# Autodesk Inventor assembly: SUBWashChamber
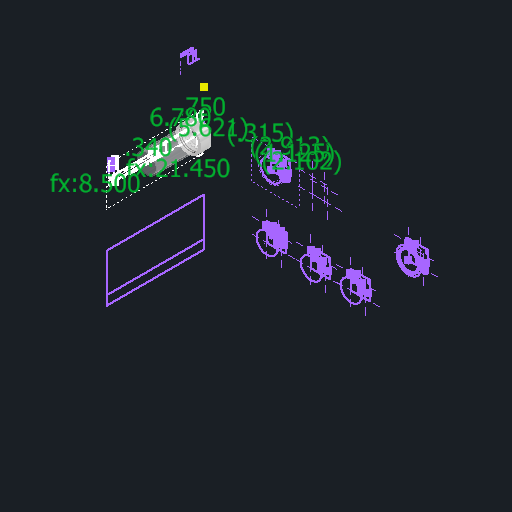
[picture p0: Inventor's stored thumbnail of the model, 512x512]
Saved by Autodesk Inventor 2024 (Build 280153000, 153)
## iProperties
Created: 2025-02-06
Part Number: SUBWashChamber
Document SubType Name: Assembly
Designer: Tommy Rohmann
Author: Tommy Rohmann
## Documents named in this file (6)
- C:\Users\Tommy Rohmann\OneDrive\Projects\Microgravity-Press-Washing-Machine\System Design and Documentation\Inventor Design Project\SUBWashChamber.iam
- C:\Users\Tommy Rohmann\OneDrive\Projects\Microgravity-Press-Washing-Machine\System Design and Documentation\Inventor Design Project\LAYOUT.ipt
- C:\Users\Tommy Rohmann\OneDrive\Projects\Microgravity-Press-Washing-Machine\System Design and Documentation\Inventor Design Project\WashChamber.ipt
- C:\Users\Tommy Rohmann\OneDrive\Projects\Microgravity-Press-Washing-Machine\System Design and Documentation\Inventor Design Project\ConduitStaticSeal.ipt
- C:\Users\Tommy Rohmann\OneDrive\Projects\Microgravity-Press-Washing-Machine\System Design and Documentation\Inventor Design Project\CastleSpacer.ipt
- C:\Users\Tommy Rohmann\OneDrive\Projects\Microgravity-Press-Washing-Machine\System Design and Documentation\Inventor Design Project\WashChamberConduit.ipt
## Components (6 placed, 5 different names)
1. LAYOUT:1
2. WashChamber:1 — Mate:6, Mate:9, Mate:11
3. ConduitStaticSeal:1 — Mate:7, Tangent:2
4. ConduitStaticSeal:2 — Mate:8, Tangent:1
5. CastleSpacer:1 — Mate:6, Mate:9, Mate:10
6. WashChamberConduit:1 — Mate:7, Mate:8, Tangent:1, Tangent:2, Mate:10, Mate:11
## Relationships (11: Mate 6, Composite 3, Tangent 2)
- [Composite]: LAYOUT:1 ↔ WashChamber:1
- [Composite]: LAYOUT:1 ↔ CastleSpacer:1
- Mate:6: WashChamber:1 ↔ CastleSpacer:1
- [Composite]: LAYOUT:1 ↔ WashChamberConduit:1
- Mate:7: ConduitStaticSeal:1 ↔ WashChamberConduit:1
- Mate:8: ConduitStaticSeal:2 ↔ WashChamberConduit:1
- Tangent:1: ConduitStaticSeal:2 ↔ WashChamberConduit:1
- Tangent:2: ConduitStaticSeal:1 ↔ WashChamberConduit:1
- Mate:9: WashChamber:1 ↔ CastleSpacer:1
- Mate:10: CastleSpacer:1 ↔ WashChamberConduit:1
- Mate:11: WashChamber:1 ↔ WashChamberConduit:1
